# Autodesk Inventor assembly: Frame With Wheels
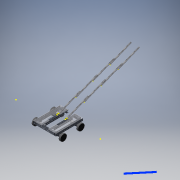
[picture p0: Inventor's stored thumbnail of the model, 180x180]
Saved by Autodesk Inventor 2016 (Build 200138000, 138)
## iProperties
Created: 2015-11-11
Part Number: Frame With Wheels
Document SubType Name: Assembly
Designer: Julia
Author: Julia
## Documents named in this file (7)
- C:\Users\jesse\Google Drive\CAD\FTC CAD Parts\Frame With Wheels.iam
- C:\Users\jesse\Google Drive\CAD\FTC CAD Parts\Robot Frame.iam
- C:\Users\jesse\Google Drive\CAD\FTC CAD Parts\Wheel mount.iam
- C:\Users\jesse\Google Drive\CAD\FTC CAD Parts\alum-uprights.ipt
- C:\Users\jesse\Google Drive\CAD\FTC CAD Parts\Andy Mark\double sided slider.ipt
- C:\Users\jesse\Google Drive\CAD\FTC CAD Parts\channel1 of lift pivot.ipt
- C:\Users\jesse\Google Drive\CAD\FTC CAD Parts\Part132.ipt
## Components (29 placed, 6 different names)
1. Wheel mount:1 [sub-assembly] — Mate:1, Mate:2, Mate:11
2. Wheel mount:2 [sub-assembly] — Mate:3, Mate:4, Mate:12
3. Wheel mount:3 [sub-assembly] — Mate:5, Mate:9, Mate:10
4. Wheel mount:4 [sub-assembly] — Mate:6, Mate:7, Mate:8
5. Robot Frame:1 [sub-assembly] — Mate:1, Mate:2, Mate:3, Mate:4, Mate:5, Mate:6, Mate:7, Mate:8, Mate:9, Mate:10, Mate:11, Mate:12, Mate:72, Angle:1, Angle:2, Mate:76, Mate:80, Mate:81
6. double sided slider:1 — Mate:48
7. alum-uprights:1 — Mate:48, Mate:75, Angle:3, Mate:77
8. double sided slider:2
9. alum-uprights:2
10. double sided slider:3
11. double sided slider:4
12. alum-uprights:3
13. double sided slider:5
14. double sided slider:6
15. alum-uprights:4 — Flush:22
16. double sided slider:7
17. alum-uprights:5 — Mate:67, Mate:68, Mate:69
18. double sided slider:8
19. alum-uprights:6
20. double sided slider:9
21. double sided slider:10
22. alum-uprights:7
23. double sided slider:11
24. double sided slider:12
25. alum-uprights:8 — Flush:22
26. channel1 of lift pivot:1 — Mate:67, Mate:68, Mate:69, Mate:70, Mate:71
27. Part132:1 — Mate:70, Mate:71, Mate:72, Angle:1, Flush:21, Mate:80
28. Part132:2 — Angle:2, Mate:76, Mate:78, Mate:79, Flush:21, Mate:81
29. channel1 of lift pivot:2 — Mate:75, Angle:3, Mate:77, Mate:78, Mate:79
## Relationships (86: Mate 61, Flush 22, Angle 3)
- Mate:1: Wheel mount:1 ↔ Robot Frame:1
- Mate:2: Wheel mount:1 ↔ Robot Frame:1
- Mate:3: Wheel mount:2 ↔ Robot Frame:1
- Mate:4: Wheel mount:2 ↔ Robot Frame:1
- Mate:5: Wheel mount:3 ↔ Robot Frame:1
- Mate:6: Wheel mount:4 ↔ Robot Frame:1
- Mate:7: Wheel mount:4 ↔ Robot Frame:1
- Mate:8: Wheel mount:4 ↔ Robot Frame:1
- Mate:9: Wheel mount:3 ↔ Robot Frame:1
- Mate:10: Wheel mount:3 ↔ Robot Frame:1
- Mate:11: Wheel mount:1 ↔ Robot Frame:1
- Mate:12: Wheel mount:2 ↔ Robot Frame:1
- [Mate]: double sided slider:1 ↔ alum-uprights:1
- [Flush]: double sided slider:1 ↔ alum-uprights:1
- [Flush]: double sided slider:2 ↔ alum-uprights:2
- [Mate]: double sided slider:2 ↔ alum-uprights:2
- [Mate]: double sided slider:2 ↔ alum-uprights:2
- [Flush]: double sided slider:1 ↔ alum-uprights:1
- [Mate]: alum-uprights:1 ↔ double sided slider:2
- [Mate]: double sided slider:1 ↔ alum-uprights:2
- [Flush]: alum-uprights:1 ↔ alum-uprights:2
- [Mate]: alum-uprights:2 ↔ double sided slider:3
- [Mate]: alum-uprights:2 ↔ double sided slider:3
- [Flush]: alum-uprights:2 ↔ double sided slider:3
- [Mate]: double sided slider:4 ↔ alum-uprights:3
- [Mate]: alum-uprights:3 ↔ double sided slider:5
- [Mate]: alum-uprights:3 ↔ double sided slider:5
- [Flush]: alum-uprights:3 ↔ double sided slider:5
- [Mate]: double sided slider:4 ↔ alum-uprights:3
- [Flush]: double sided slider:4 ↔ alum-uprights:3
- [Mate]: double sided slider:6 ↔ alum-uprights:4
- [Mate]: double sided slider:6 ↔ alum-uprights:4
- [Flush]: double sided slider:6 ↔ alum-uprights:4
- [Mate]: alum-uprights:2 ↔ double sided slider:4
- [Mate]: alum-uprights:2 ↔ double sided slider:4
- [Flush]: alum-uprights:2 ↔ alum-uprights:3
- [Mate]: alum-uprights:3 ↔ double sided slider:6
- [Mate]: alum-uprights:3 ↔ double sided slider:6
- [Flush]: alum-uprights:3 ↔ alum-uprights:4
- Mate:48: double sided slider:1 ↔ alum-uprights:1
- [Mate]: double sided slider:7 ↔ alum-uprights:5
- [Flush]: double sided slider:7 ↔ alum-uprights:5
- [Flush]: double sided slider:8 ↔ alum-uprights:6
- [Mate]: double sided slider:8 ↔ alum-uprights:6
- [Mate]: double sided slider:8 ↔ alum-uprights:6
- [Flush]: double sided slider:7 ↔ alum-uprights:5
- [Mate]: alum-uprights:5 ↔ double sided slider:8
- [Mate]: double sided slider:7 ↔ alum-uprights:6
- [Flush]: alum-uprights:5 ↔ alum-uprights:6
- [Mate]: alum-uprights:6 ↔ double sided slider:9
- [Mate]: alum-uprights:6 ↔ double sided slider:9
- [Flush]: alum-uprights:6 ↔ double sided slider:9
- [Mate]: double sided slider:10 ↔ alum-uprights:7
- [Mate]: alum-uprights:7 ↔ double sided slider:11
- [Mate]: alum-uprights:7 ↔ double sided slider:11
- [Flush]: alum-uprights:7 ↔ double sided slider:11
- [Mate]: double sided slider:10 ↔ alum-uprights:7
- [Flush]: double sided slider:10 ↔ alum-uprights:7
- [Mate]: double sided slider:12 ↔ alum-uprights:8
- [Mate]: double sided slider:12 ↔ alum-uprights:8
- [Flush]: double sided slider:12 ↔ alum-uprights:8
- [Mate]: alum-uprights:6 ↔ double sided slider:10
- [Mate]: alum-uprights:6 ↔ double sided slider:10
- [Flush]: alum-uprights:6 ↔ alum-uprights:7
- [Mate]: alum-uprights:7 ↔ double sided slider:12
- [Mate]: alum-uprights:7 ↔ double sided slider:12
- [Flush]: alum-uprights:7 ↔ alum-uprights:8
- [Mate]: double sided slider:7 ↔ alum-uprights:5
- Mate:67: alum-uprights:5 ↔ channel1 of lift pivot:1
- Mate:68: alum-uprights:5 ↔ channel1 of lift pivot:1
- Mate:69: alum-uprights:5 ↔ channel1 of lift pivot:1
- Mate:70: channel1 of lift pivot:1 ↔ Part132:1
- Mate:71: channel1 of lift pivot:1 ↔ Part132:1
- Mate:72: Robot Frame:1 ↔ Part132:1
- Mate:75: alum-uprights:1 ↔ channel1 of lift pivot:2
- Angle:1 (0 deg): Robot Frame:1 ↔ Part132:1
- Angle:2 (0 deg): Robot Frame:1 ↔ Part132:2
- Mate:76: Robot Frame:1 ↔ Part132:2
- Angle:3 (0 deg): alum-uprights:1 ↔ channel1 of lift pivot:2
- Mate:77: alum-uprights:1 ↔ channel1 of lift pivot:2
- Mate:78: Part132:2 ↔ channel1 of lift pivot:2
- Mate:79: Part132:2 ↔ channel1 of lift pivot:2
- Flush:21: Part132:1 ↔ Part132:2
- Flush:22: alum-uprights:4 ↔ alum-uprights:8
- Mate:80 (0.762 mm): Robot Frame:1 ↔ Part132:1
- Mate:81 (0.5334 mm): Robot Frame:1 ↔ Part132:2
## Named parameters: d35_d0 = 0 mm, d36_d1 = 0 mm, d37_d39 = 275.59 mm, d38_d40 = 0 mm, d39_d41 = 0 mm, d40_d42 = 0 mm, d41_d43 = 0 mm, d42_d44 = 275.59 mm, d43_d45 = 0 mm, d20_d19 = 0 mm, d21_d17 = 0 mm, d22_d18 = 0 mm, d23_d11 = 0 mm, d33_d23_d11 = 0 mm, d34_d28 = 0 mm, d35_d29 = 0 mm, d62_d6 = 0 mm, d63_d7 = 0 mm, d64_d8 = 0 mm, d65_d9 = 0 mm, d66_d10 = 0 mm, d67_d11 = 0 mm, d104_d103 = 0 mm, d105_d35_d0 = 0 mm, d106_d36_d1 = 0 mm, d107_d37_d39 = 275.59 mm, d108_d38_d40 = 0 mm, d109_d39_d41 = 0 mm, d110_d40_d42 = 0 mm, d111_d41_d43 = 0 mm, d112_d42_d44 = 275.59 mm, d113_d43_d45 = 0 mm, d114_d19 = 0 mm, d115_d20_d19 = 0 mm, d116_d21_d17 = 0 mm, d117_d22_d18 = 0 mm, d118_d23_d11 = 0 mm, d119_d28 = 0 mm, d120_d29 = 0 mm, d121_d33_d23_d11 = 0 mm, d122_d34_d28 = 0 mm, d123_d35_d29 = 0 mm, d124_d36 = 0 mm, d125_d37 = 0 mm, d126_d38 = 0 mm, d127_d14 = 0 mm, d128_d15 = 275.59 mm, d129_d16 = 0 mm, d130_d17 = 0 mm, d131_d18 = 0 mm, d132_d62_d6 = 0 mm, d133_d63_d7 = 0 mm, d134_d64_d8 = 0 mm, d135_d65_d9 = 0 mm, d136_d66_d10 = 0 mm, d137_d67_d11 = 0 mm
